# Autodesk Inventor assembly: HDzero nano with micro spacer assy
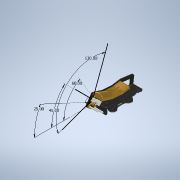
[picture p0: Inventor's stored thumbnail of the model, 180x180]
Saved by Autodesk Inventor 2020 (Build 240168000, 168)
## iProperties
Created: 2022-05-03
Part Number: HDzero nano with micro spacer assy
Document SubType Name: Assembly
Designer: Steven
Author: Steven
## Documents named in this file (8)
- Y:\FPV drone stuff\0 Street League\Frames\PB-Kauri-X\3D prints\35 mm canopy\work in progress prints\HDzero nano with micro spacer assy.iam
- Y:\FPV drone stuff\0 Street League\Frames\PB-Kauri-X\Kauri side plate.ipt
- Y:\FPV drone stuff\0 Street League\Frames\PB-Kauri-X\3D prints\35 mm canopy\KauriCanopy Pb.ipt
- Y:\FPV drone stuff\0 Street League\Frames\PB-Kauri-X\Kauri mid plate v2.ipt
- Y:\FPV drone stuff\0 Street League\Frames\PB-Kauri-X\3D prints\35 mm canopy\KauriFrontLink 35mm.ipt
- Y:\FPV drone stuff\0 Street League\Frames\PB-Kauri-X\3D prints\35 mm canopy\KauriRearLink 35mm no brass insert.ipt
- Y:\FPV drone stuff\0 Street League\Frames\PB-Kauri-X\3D prints\35 mm canopy\35mm standoff.ipt
- Y:\FPV drone stuff\0 Street League\Frames\PB-Kauri-X\3D prints\35 mm canopy\work in progress prints\nano cam assy.iam
## Components (9 placed, 7 different names)
1. Kauri side plate:1 — Insert:2, Insert:4, Insert:5, Insert:6
2. Kauri side plate:2 — Insert:1, Insert:3, Insert:9, Insert:10, Mate:3, Mate:8
3. KauriCanopy Pb:1 — Insert:1, Insert:2, Insert:3, Insert:4
4. KauriFrontLink 35mm:1 — Insert:5, Flush:1, Mate:1, Insert:7
5. KauriRearLink 35mm no brass insert:1 — Insert:6, Flush:1, Insert:8
6. Kauri mid plate v2:1 — Mate:1, Insert:7, Insert:8, Mate:7
7. 35mm standoff:1 — Insert:9, Mate:10
8. 35mm standoff:2 — Insert:10, Mate:9
9. nano cam assy:1 [sub-assembly] — Mate:8, Mate:9, Mate:10
## Relationships (17: Insert 10, Mate 6, Flush 1)
- Insert:1: Kauri side plate:2 ↔ KauriCanopy Pb:1
- Insert:2: Kauri side plate:1 ↔ KauriCanopy Pb:1
- Insert:3: Kauri side plate:2 ↔ KauriCanopy Pb:1
- Insert:4: Kauri side plate:1 ↔ KauriCanopy Pb:1
- Insert:5: Kauri side plate:1 ↔ KauriFrontLink 35mm:1
- Insert:6: Kauri side plate:1 ↔ KauriRearLink 35mm no brass insert:1
- Flush:1: KauriFrontLink 35mm:1 ↔ KauriRearLink 35mm no brass insert:1
- Mate:1: KauriFrontLink 35mm:1 ↔ Kauri mid plate v2:1
- Insert:7: KauriFrontLink 35mm:1 ↔ Kauri mid plate v2:1
- Insert:8: KauriRearLink 35mm no brass insert:1 ↔ Kauri mid plate v2:1
- Insert:9: Kauri side plate:2 ↔ 35mm standoff:1
- Insert:10: Kauri side plate:2 ↔ 35mm standoff:2
- Mate:3: Kauri side plate:2
- Mate:7: Kauri mid plate v2:1
- Mate:8: Kauri side plate:2 ↔ nano cam assy:1
- Mate:9: 35mm standoff:2 ↔ nano cam assy:1
- Mate:10: 35mm standoff:1 ↔ nano cam assy:1
